# Autodesk Inventor assembly: 組合1
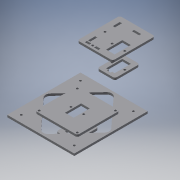
[picture p0: Inventor's stored thumbnail of the model, 180x180]
Saved by Autodesk Inventor 2017 (Build 210142000, 142)
## iProperties
Part Number: 組合1
Material: 一般
Document SubType Name: Assembly
Designer: User
Author: User
## Documents named in this file (5)
- C:\Users\User\Desktop\專題\零件\組合1.iam
- C:\Users\User\Desktop\專題\零件\板子3.ipt
- C:\Users\User\Desktop\專題\零件\板子5.ipt
- C:\Users\User\Desktop\專題\零件\板子4.ipt
- C:\Users\User\Desktop\專題\零件\板子1.ipt
## Components (5 placed, 4 different names)
1. 板子3:1 — 插入:1, 插入:2
2. 板子5:1 — 插入:1, 插入:2, 插入:3, 插入:4
3. 板子4:1 — 插入:3, 插入:4
4. 板子1:1 — 插入:5, 插入:6
5. 板子4:2 — 插入:5, 插入:6
## Relationships (6: Insert 6)
- 插入:1 [Insert]: 板子3:1 ↔ 板子5:1
- 插入:2 [Insert]: 板子3:1 ↔ 板子5:1
- 插入:3 [Insert] (20 mm): 板子5:1 ↔ 板子4:1
- 插入:4 [Insert] (20 mm): 板子5:1 ↔ 板子4:1
- 插入:5 [Insert] (20 mm): 板子1:1 ↔ 板子4:2
- 插入:6 [Insert] (20 mm): 板子1:1 ↔ 板子4:2
